# Autodesk Inventor assembly: Tablet-Halterung Nacharbeit
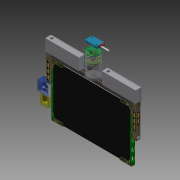
[picture p0: Inventor's stored thumbnail of the model, 180x180]
Saved by Autodesk Inventor 2014 SP1 (Build 180222100, 222)
## iProperties
Created: 2013-08-01
Part Number: Tablet-Halterung Nacharbeit
Document SubType Name: Assembly
Designer: vogel
Author: vogel
## Documents named in this file (59)
- Z:\131087 - Tablet-Halterung\Tablet-Halterung Nacharbeit.iam
- Z:\131087 - Tablet-Halterung\13_1087_001.ipt
- Z:\131087 - Tablet-Halterung\Tablet - Nexus 10.ipt
- Z:\131087 - Tablet-Halterung\13_1087_003.ipt
- Z:\131087 - Tablet-Halterung\13_1087_004.ipt
- C:\Users\vogel.WWF-AD\Documents\Inventor\Content Center Files\R2014\de-DE\ISO 8734(2)\ISO 8734 - 2 x 12 - AISO (2).ipt
- Z:\131087 - Tablet-Halterung\13_1087_005.ipt
- Z:\131087 - Tablet-Halterung\13_1087_002.ipt
- Z:\131087 - Tablet-Halterung\13_1087_007.ipt
- Z:\131087 - Tablet-Halterung\Getriebe.iam
- Z:\131087 - Tablet-Halterung\13_1087_008.ipt
- Z:\131087 - Tablet-Halterung\13_1087_009.ipt
- Z:\131087 - Tablet-Halterung\Sinterbuchse 35 60 325 48106.ipt
- Z:\131087 - Tablet-Halterung\13_1087_016.ipt
- Z:\131087 - Tablet-Halterung\13_1087_017.ipt
- Z:\131087 - Tablet-Halterung\IOIO Board.ipt
- Z:\131087 - Tablet-Halterung\13_1087_018.ipt
- Z:\131087 - Tablet-Halterung\13_1087_019.ipt
- C:\Users\vogel.WWF-AD\Documents\Inventor\Content Center Files\R2014\de-DE\ISO 4026\ISO 4026 - M3 x 5ISO.ipt
- Z:\131087 - Tablet-Halterung\13_1087_020.ipt
- Z:\131087 - Tablet-Halterung\Akku.ipt
- Z:\131087 - Tablet-Halterung\Platine.ipt
- Z:\131087 - Tablet-Halterung\13_0204_040.ipt
- Z:\131087 - Tablet-Halterung\13_1087_023.ipt
- Z:\131087 - Tablet-Halterung\13_1087_024.ipt
- Z:\131087 - Tablet-Halterung\Motor XDRIVE GM12F.ipt
- Z:\131087 - Tablet-Halterung\13_1087_025.ipt
- Z:\131087 - Tablet-Halterung\13_1087_027.ipt
- Z:\131087 - Tablet-Halterung\13_1087_028.ipt
- Z:\131087 - Tablet-Halterung\13_1087_029.ipt
- Z:\131087 - Tablet-Halterung\13_1087_030.ipt
- Z:\131087 - Tablet-Halterung\13_1087_032.ipt
- Z:\131087 - Tablet-Halterung\Sinterbuchse 35 60 325 61014.ipt
- C:\Users\vogel.WWF-AD\Documents\Inventor\Content Center Files\R2014\de-DE\ISO 8734(2)\ISO 8734 - 3 x 8 - AISO (2).ipt
- Z:\131087 - Tablet-Halterung\13_1087_034.ipt
- Z:\131087 - Tablet-Halterung\13_1087_035.ipt
- Z:\131087 - Tablet-Halterung\13_1087_036.ipt
- Z:\131087 - Tablet-Halterung\13_1087_037.ipt
- Z:\131087 - Tablet-Halterung\13_1087_038.ipt
- Z:\131087 - Tablet-Halterung\13_1087_039.ipt
- Z:\131087 - Tablet-Halterung\13_1087_040.ipt
- C:\Users\vogel.WWF-AD\Documents\Inventor\Content Center Files\R2014\de-DE\ISO 2009(2)\ISO 2009 - M2 x 6ISO 4.ipt
- C:\Users\vogel.WWF-AD\Documents\Inventor\Content Center Files\R2014\de-DE\ISO 2009(2)\ISO 2009 - M3 x 6ISO 3,35.ipt
- C:\Users\vogel.WWF-AD\Documents\Inventor\Content Center Files\R2014\de-DE\ISO 10642(1)\ISO 10642 - M3 x  10.ipt
- Z:\131087 - Tablet-Halterung\13_1087_041.ipt
- C:\Users\vogel.WWF-AD\Documents\Inventor\Content Center Files\R2014\de-DE\ISO 2009(2)\ISO 2009 - M2 x 12ISO 10.ipt
- C:\Users\vogel.WWF-AD\Documents\Inventor\Content Center Files\R2014\de-DE\ISO 10642(1)\ISO 10642 - M3 x  16.ipt
- C:\Users\vogel.WWF-AD\Documents\Inventor\Content Center Files\R2014\de-DE\ISO 2009(2)\ISO 2009 - M2 x 3ISO 1.ipt
- C:\Users\vogel.WWF-AD\Documents\Inventor\Content Center Files\R2014\de-DE\ISO 1207(2)\ISO 1207 - M1,6 x 6.ipt
- C:\Users\vogel.WWF-AD\Documents\Inventor\Content Center Files\R2014\de-DE\DIN 6799\DIN 6799 - 2,3 3.ipt
- C:\Users\vogel.WWF-AD\Documents\Inventor\Content Center Files\R2014\de-DE\ISO 4762(2)\ISO 4762 - M4 x 12ISO.ipt
- C:\Users\vogel.WWF-AD\Documents\Inventor\Content Center Files\R2014\de-DE\ISO 4766(1)\ISO 4766 - M2 x 2DIN EN.ipt
- C:\Users\vogel.WWF-AD\Documents\Inventor\Content Center Files\R2014\de-DE\ISO 10642(1)\ISO 10642 - M3 x  8.ipt
- Z:\131087 - Tablet-Halterung\13_1087_042.ipt
- C:\Users\vogel.WWF-AD\Documents\Inventor\Content Center Files\R2014\de-DE\DIN 471(3)\DIN 471 - 4 x 0,4.ipt
- Z:\131087 - Tablet-Halterung\Zahnräder mädler 21401200.ipt
- C:\Users\vogel.WWF-AD\Documents\Inventor\Content Center Files\R2014\de-DE\ISO 4026\ISO 4026 - M3 x 3ISO.ipt
- Z:\131087 - Tablet-Halterung\13_1087_060.ipt
- Z:\131087 - Tablet-Halterung\13_1087_061.ipt
## Components (124 placed, 58 different names)
1. 13_1087_001:1 — Passend:2, Fluchtend:2, Passend:8, Passend:40, Passend:132
2. Tablet - Nexus 10:1 — Passend:2, Passend:5, Passend:9, Passend:10, Fluchtend:7
3. 13_1087_001:2 — Einfügen:2, Passend:11, Passend:130
4. 13_1087_001:3 — Passend:5, Passend:6, Passend:7, Fluchtend:1, Passend:131
5. 13_1087_003:1 — Passend:6, Passend:7, Fluchtend:1, Einfügen:1, Winkel:1, Passend:9, Fluchtend:3, Fluchtend:4, Einfügen:10, Passend:24, Einfügen:12, Passend:39
6. 13_1087_004:1 — Fluchtend:2, Verschiebbar:1, Passend:8, Passend:40
7. 13_1087_005:1 — Passend:10, Fluchtend:3, Fluchtend:4, Einfügen:2, Passend:11, Passend:12, Passend:13, Fluchtend:5, Einfügen:3, Passend:67, Passend:88, Passend:117, Fluchtend:29
8. 13_1087_004:2 — Passend:12, Passend:13, Fluchtend:5, Einfügen:4, Passend:14
9. 13_1087_002:1 — Einfügen:4, Passend:14, Passend:133
10. 13_1087_007:1 — Fluchtend:7, Passend:22, Einfügen:7, Fluchtend:8, Einfügen:14, Passend:59, Passend:94, Passend:95, Passend:102, Passend:103, Passend:104, Passend:105, Passend:115, Passend:116, Achse 1, Einfügen:73, Passend:166
11. 13_1087_016:1 — Passend:24, Einfügen:12, Passend:38, Einfügen:39, Achse 2, Einfügen:72
12. Getriebe:1 [sub-assembly] — Passend:37, Passend:66, Passend:67, Passend:99
13. 13_1087_008:1 — Fluchtend:8, Einfügen:14, Fluchtend:9, Fluchtend:10, Fluchtend:11, Passend:28, Passend:29, Passend:30, Passend:31, Passend:32, Passend:33, Passend:37, Passend:66, Passend:96, Passend:97, Passend:98, Passend:114, Fluchtend:32
14. 13_1087_009:1 — Passend:22, Einfügen:7, Einfügen:8, Passend:34, Passend:35, Passend:36, Achse 2, Passend:41, Passend:42, Passend:43, Passend:44, Passend:45, Passend:46, Fluchtend:21, Passend:107, Passend:108, Passend:109, Einfügen:71, Fluchtend:31
15. Sinterbuchse 35 60 325 48106:1 — Einfügen:8, Einfügen:39
16. 13_1087_017:1 — Einfügen:10, Fluchtend:28
17. IOIO Board:1 — Passend:57, Passend:58, Passend:76
18. 13_1087_018:1 — Fluchtend:9, Passend:28, Passend:29, Passend:122, Passend:123, Einfügen:62, Einfügen:65
19. 13_1087_019:1 — Fluchtend:10, Passend:30, Passend:31, Einfügen:20, Einfügen:23, Passend:120, Passend:121
20. 13_1087_018:2 — Fluchtend:11, Passend:32, Passend:33, Passend:118, Passend:119, Einfügen:60, Einfügen:63
21. 13_1087_018:3 — Passend:34, Passend:35, Passend:36, Einfügen:50, Einfügen:51, Passend:124, Passend:125
22. 13_1087_019:2 — Passend:41, Passend:42, Passend:43, Einfügen:16, Einfügen:17, Passend:126, Passend:127
23. 13_1087_018:4 — Passend:44, Passend:45, Passend:46, Passend:128, Passend:129, Einfügen:58, Einfügen:59
24. Akku:1 — Passend:50, Passend:51, Passend:52
25. 13_1087_017:2 — Passend:88, Fluchtend:28
26. Platine:1 — Passend:54, Passend:77, Passend:78
27. 13_0204_040:1 — Einfügen:43, Einfügen:44, Achse 1
28. 13_1087_023:1 — Fluchtend:15, Fluchtend:16, Passend:49, Passend:50, Passend:51, Passend:52, Fluchtend:20, Fluchtend:21, Fluchtend:22, Fluchtend:32
29. 13_1087_024:1 — Fluchtend:15, Fluchtend:16, Passend:49, Passend:144, Passend:145, Passend:146, Passend:147
30. 13_1087_023:2 — Passend:54, Passend:57, Passend:58, Fluchtend:20, Einfügen:30, Einfügen:31, Passend:59, Fluchtend:22, Passend:76, Passend:77, Passend:78, Passend:91, Passend:92, Passend:93, Fluchtend:31
31. 13_1087_024:2 — Einfügen:30, Einfügen:31, Passend:140, Passend:141, Passend:142, Passend:143
32. Motor XDRIVE GM12F:1 — Einfügen:34, Einfügen:41, Passend:153
33. 13_1087_025:1 — Einfügen:46, Passend:165, Einfügen:76
34. 13_1087_027:1 — Einfügen:34, Passend:72, Passend:154, Passend:159, Passend:160
35. 13_1087_030:1 — Passend:72, Einfügen:41, Einfügen:45, Passend:86, Einfügen:53, Einfügen:54, Einfügen:66, Einfügen:67, Einfügen:74, Passend:167, Passend:168
36. 13_1087_032:1 — Einfügen:43, Einfügen:44, Einfügen:49, Passend:82, Passend:83, Einfügen:52, Fluchtend:26, Passend:84, Einfügen:55, Einfügen:56
37. Sinterbuchse 35 60 325 61014:1 — Einfügen:45, Einfügen:46
38. 13_1087_034:1 — Passend:82, Passend:83
39. 13_1087_035:1 — Einfügen:52, Passend:85, Passend:139
40. 13_1087_036:1 — Fluchtend:26, Passend:84, Passend:85, Passend:155
41. 13_1087_037:1 — Passend:86, Passend:137, Passend:138, Einfügen:66, Einfügen:67
42. 13_1087_038:1 — Passend:91, Passend:92, Passend:93, Passend:100, Passend:101
43. 13_1087_039:1 — Passend:94, Passend:95, Passend:96, Passend:148, Passend:149
44. 13_1087_040:1 — Passend:97, Passend:98, Passend:99, Passend:112, Passend:113
45. 13_1087_041:1 — Passend:107, Passend:108, Passend:109, Passend:110, Passend:111
46. ISO 8734 2 x 12 - A:1 — Einfügen:1, Winkel:1, Verschiebbar:1
47. ISO 8734 2 x 12 - A:2 — Einfügen:3
48. ISO 4026 M3 x 5:1 — Passend:38, Passend:39
49. ISO 8734 3 x 8 - A:1 — Einfügen:49
50. ISO 2009 M2 x 6 x 4:1 — Passend:100
51. ISO 2009 M2 x 6 x 4:2 — Passend:101
52. ISO 2009 M3 x 6 x 3,35:1 — Passend:102
53. ISO 2009 M3 x 6 x 3,35:2 — Passend:103
54. ISO 2009 M3 x 6 x 3,35:3 — Passend:104
55. ISO 2009 M3 x 6 x 3,35:4 — Passend:105
56. ISO 2009 M2 x 12 x 10:1 — Passend:110
57. ISO 2009 M2 x 12 x 10:2 — Passend:111
58. ISO 2009 M2 x 12 x 10:3 — Passend:112
59. ISO 2009 M2 x 12 x 10:4 — Passend:113
60. ISO 10642 M3 x  10:2 — Passend:114
61. ISO 10642 M3 x  16:1 — Passend:115
62. ISO 10642 M3 x  16:2 — Passend:116
63. ISO 4026 M3 x 5:2 — Passend:117, Fluchtend:29
64. ISO 2009 M2 x 3 x 1:1 — Passend:118
65. ISO 2009 M2 x 3 x 1:2 — Passend:119
66. ISO 2009 M2 x 3 x 1:3 — Passend:120
67. ISO 2009 M2 x 3 x 1:4 — Passend:121
68. ISO 2009 M2 x 3 x 1:5 — Passend:122
69. ISO 2009 M2 x 3 x 1:6 — Passend:123
70. ISO 2009 M2 x 3 x 1:7 — Passend:124
71. ISO 2009 M2 x 3 x 1:8 — Passend:125
72. ISO 2009 M2 x 3 x 1:9 — Passend:126
73. ISO 2009 M2 x 3 x 1:10 — Passend:127
74. ISO 2009 M2 x 3 x 1:11 — Passend:128
75. ISO 2009 M2 x 3 x 1:12 — Passend:129
76. ISO 2009 M2 x 6 x 4:3 — Passend:130
77. ISO 2009 M2 x 6 x 4:4 — Passend:131
78. ISO 2009 M2 x 6 x 4:5 — Passend:132
79. ISO 2009 M2 x 6 x 4:6 — Passend:133
80. ISO 10642 M3 x  10:3 — Passend:137
81. ISO 10642 M3 x  10:4 — Passend:138
82. ISO 1207 M1,6 x 6:1 — Einfügen:53
83. ISO 1207 M1,6 x 6:2 — Einfügen:54
84. DIN 6799 2,3:1 — Passend:139
85. ISO 4762 M4 x 12:1 — Einfügen:55
86. ISO 4762 M4 x 12:2 — Einfügen:56
87. ISO 2009 M2 x 6 x 4:7 — Passend:140
88. ISO 2009 M2 x 6 x 4:8 — Passend:141
89. ISO 2009 M2 x 6 x 4:9 — Passend:142
90. ISO 2009 M2 x 6 x 4:10 — Passend:143
91. ISO 2009 M2 x 6 x 4:11 — Passend:144
92. ISO 2009 M2 x 6 x 4:12 — Passend:145
93. ISO 2009 M2 x 6 x 4:13 — Passend:146
94. ISO 2009 M2 x 6 x 4:14 — Passend:147
95. ISO 2009 M2 x 12 x 10:5 — Passend:148
96. ISO 2009 M2 x 12 x 10:6 — Passend:149
97. DIN EN 24766 M2 x 2:1 — Passend:153, Passend:154
98. ISO 10642 M3 x  8:1 — Passend:155
99. 13_1087_042:1 — Einfügen:71
100. DIN 471 <= 9mm 4 x 0,4:1 — Einfügen:72
101. Zahnräder mädler 21401200:1 — Passend:159, Passend:160, Fluchtend:30, Passend:161, Passend:162
102. Zahnräder mädler 21401200:2 — Fluchtend:30, Passend:163, Passend:164, Passend:165
103. ISO 4026 M3 x 3:1 — Passend:161, Passend:162
104. ISO 4026 M3 x 3:2 — Passend:163, Passend:164
105. 13_1087_060:1 — Einfügen:73, Passend:166, Einfügen:74, Passend:167, Einfügen:75
106. 13_1087_028:1 — Einfügen:76, Einfügen:77
107. 13_1087_029:1 — Einfügen:75, Passend:168
108. 13_1087_061:1 — Einfügen:77
109. 13_1087_020:3 — Einfügen:20, Einfügen:23
110. 13_1087_020:9
111. 13_1087_020:5 — Einfügen:16, Einfügen:17
112. 13_1087_020:14
113. 13_1087_020:22 — Einfügen:62, Einfügen:65
114. 13_1087_020:20 — Einfügen:60, Einfügen:63
115. 13_1087_020:19 — Einfügen:58, Einfügen:59
116. 13_1087_020:17 — Einfügen:50, Einfügen:51
117. 13_1087_020:25
118. 13_1087_020:26
119. 13_1087_020:27
120. 13_1087_020:28
121. 13_1087_020:29
122. 13_1087_020:30
123. 13_1087_020:31
124. 13_1087_020:32
## Component patterns: (2 elements, first: 13_1087_020:3), (2 elements, first: 13_1087_020:5), (3 elements, first: 13_1087_020:22 + 13_1087_020:20 + 13_1087_020:19 + 13_1087_020:17)
## Relationships (190: Mate 120, Insert 45, Flush 21, Angle 3, TranslationJoint 1)
- Passend:2 [Mate]: 13_1087_001:1 ↔ Tablet - Nexus 10:1
- Passend:5 [Mate]: Tablet - Nexus 10:1 ↔ 13_1087_001:3
- Passend:6 [Mate]: 13_1087_001:3 ↔ 13_1087_003:1
- Passend:7 [Mate]: 13_1087_001:3 ↔ 13_1087_003:1
- Fluchtend:1 [Flush]: 13_1087_001:3 ↔ 13_1087_003:1
- Fluchtend:2 [Flush]: 13_1087_001:1 ↔ 13_1087_004:1
- Einfügen:1 [Insert]: 13_1087_003:1 ↔ ISO 8734 2 x 12 - A:1
- Winkel:1 [Angle] (90 deg): 13_1087_003:1 ↔ ISO 8734 2 x 12 - A:1
- Verschiebbar:1 [TranslationJoint]: 13_1087_004:1 ↔ ISO 8734 2 x 12 - A:1
- Passend:8 [Mate]: 13_1087_001:1 ↔ 13_1087_004:1
- Passend:9 [Mate] (0.1 mm): Tablet - Nexus 10:1 ↔ 13_1087_003:1
- Passend:10 [Mate] (0.1 mm): Tablet - Nexus 10:1 ↔ 13_1087_005:1
- Fluchtend:3 [Flush]: 13_1087_003:1 ↔ 13_1087_005:1
- Fluchtend:4 [Flush]: 13_1087_003:1 ↔ 13_1087_005:1
- Einfügen:2 [Insert]: 13_1087_001:2 ↔ 13_1087_005:1
- Passend:11 [Mate]: 13_1087_001:2 ↔ 13_1087_005:1
- Passend:12 [Mate]: 13_1087_005:1 ↔ 13_1087_004:2
- Passend:13 [Mate]: 13_1087_005:1 ↔ 13_1087_004:2
- Fluchtend:5 [Flush]: 13_1087_005:1 ↔ 13_1087_004:2
- Einfügen:3 [Insert]: 13_1087_005:1 ↔ ISO 8734 2 x 12 - A:2
- Einfügen:4 [Insert]: 13_1087_004:2 ↔ 13_1087_002:1
- Passend:14 [Mate]: 13_1087_004:2 ↔ 13_1087_002:1
- Fluchtend:7 [Flush]: Tablet - Nexus 10:1 ↔ 13_1087_007:1
- Passend:22 [Mate]: 13_1087_007:1 ↔ 13_1087_009:1
- Einfügen:7 [Insert]: 13_1087_007:1 ↔ 13_1087_009:1
- Einfügen:8 [Insert]: 13_1087_009:1 ↔ Sinterbuchse 35 60 325 48106:1
- Einfügen:10 [Insert]: 13_1087_003:1 ↔ 13_1087_017:1
- Passend:24 [Mate]: 13_1087_003:1 ↔ 13_1087_016:1
- Einfügen:12 [Insert] (1.5 mm): 13_1087_003:1 ↔ 13_1087_016:1
- Fluchtend:8 [Flush]: 13_1087_007:1 ↔ 13_1087_008:1
- Einfügen:14 [Insert]: 13_1087_007:1 ↔ 13_1087_008:1
- Fluchtend:9 [Flush] (-3.5 mm): 13_1087_008:1 ↔ 13_1087_018:1
- Fluchtend:10 [Flush] (3.5 mm): 13_1087_008:1 ↔ 13_1087_019:1
- Fluchtend:11 [Flush] (-3.5 mm): 13_1087_008:1 ↔ 13_1087_018:2
- Passend:28 [Mate]: 13_1087_008:1 ↔ 13_1087_018:1
- Passend:29 [Mate]: 13_1087_008:1 ↔ 13_1087_018:1
- Passend:30 [Mate]: 13_1087_008:1 ↔ 13_1087_019:1
- Passend:31 [Mate]: 13_1087_008:1 ↔ 13_1087_019:1
- Passend:32 [Mate]: 13_1087_008:1 ↔ 13_1087_018:2
- Passend:33 [Mate]: 13_1087_008:1 ↔ 13_1087_018:2
- Passend:34 [Mate]: 13_1087_009:1 ↔ 13_1087_018:3
- Passend:35 [Mate]: 13_1087_009:1 ↔ 13_1087_018:3
- Passend:36 [Mate]: 13_1087_009:1 ↔ 13_1087_018:3
- Passend:37 [Mate]: Getriebe:1 ↔ 13_1087_008:1
- Passend:38 [Mate]: 13_1087_016:1 ↔ ISO 4026 M3 x 5:1
- Passend:39 [Mate]: 13_1087_003:1 ↔ ISO 4026 M3 x 5:1
- Passend:40 [Mate]: 13_1087_001:1 ↔ 13_1087_004:1
- Passend:41 [Mate]: 13_1087_009:1 ↔ 13_1087_019:2
- Passend:42 [Mate]: 13_1087_009:1 ↔ 13_1087_019:2
- Passend:43 [Mate]: 13_1087_009:1 ↔ 13_1087_019:2
- Passend:44 [Mate]: 13_1087_009:1 ↔ 13_1087_018:4
- Passend:45 [Mate]: 13_1087_009:1 ↔ 13_1087_018:4
- Passend:46 [Mate]: 13_1087_009:1 ↔ 13_1087_018:4
- Einfügen:16 [Insert]: 13_1087_019:2 ↔ 13_1087_020:5
- Einfügen:17 [Insert]: 13_1087_019:2 ↔ 13_1087_020:5
- Einfügen:20 [Insert]: 13_1087_019:1 ↔ 13_1087_020:3
- Einfügen:23 [Insert]: 13_1087_019:1 ↔ 13_1087_020:3
- Fluchtend:15 [Flush]: 13_1087_023:1 ↔ 13_1087_024:1
- Fluchtend:16 [Flush]: 13_1087_023:1 ↔ 13_1087_024:1
- Passend:49 [Mate]: 13_1087_023:1 ↔ 13_1087_024:1
- Passend:50 [Mate]: Akku:1 ↔ 13_1087_023:1
- Passend:51 [Mate]: Akku:1 ↔ 13_1087_023:1
- Passend:52 [Mate]: Akku:1 ↔ 13_1087_023:1
- Passend:54 [Mate] (4 mm): Platine:1 ↔ 13_1087_023:2
- Passend:57 [Mate] (4 mm): IOIO Board:1 ↔ 13_1087_023:2
- Passend:58 [Mate] (5 mm): IOIO Board:1 ↔ 13_1087_023:2
- Fluchtend:20 [Flush]: 13_1087_023:1 ↔ 13_1087_023:2
- Einfügen:30 [Insert]: 13_1087_023:2 ↔ 13_1087_024:2
- Einfügen:31 [Insert]: 13_1087_023:2 ↔ 13_1087_024:2
- Passend:59 [Mate]: 13_1087_007:1 ↔ 13_1087_023:2
- Fluchtend:21 [Flush] (-3 mm): 13_1087_009:1 ↔ 13_1087_023:1
- Fluchtend:22 [Flush]: 13_1087_023:1 ↔ 13_1087_023:2
- Passend:66 [Mate]: Getriebe:1 ↔ 13_1087_008:1
- Passend:67 [Mate]: 13_1087_005:1 ↔ Getriebe:1
- Einfügen:34 [Insert] (-3.5 mm): Motor XDRIVE GM12F:1 ↔ 13_1087_027:1
- Passend:72 [Mate]: 13_1087_027:1 ↔ 13_1087_030:1
- Einfügen:39 [Insert]: 13_1087_016:1 ↔ Sinterbuchse 35 60 325 48106:1
- Achse 2 [Angle] (180 deg): 13_1087_016:1 ↔ 13_1087_009:1
- Einfügen:41 [Insert]: Motor XDRIVE GM12F:1 ↔ 13_1087_030:1
- Einfügen:43 [Insert]: 13_0204_040:1 ↔ 13_1087_032:1
- Einfügen:44 [Insert]: 13_0204_040:1 ↔ 13_1087_032:1
- Passend:76 [Mate] (2.5 mm): IOIO Board:1 ↔ 13_1087_023:2
- Passend:77 [Mate]: Platine:1 ↔ 13_1087_023:2
- Passend:78 [Mate] (5 mm): Platine:1 ↔ 13_1087_023:2
- Einfügen:45 [Insert]: 13_1087_030:1 ↔ Sinterbuchse 35 60 325 61014:1
- Einfügen:46 [Insert]: 13_1087_025:1 ↔ Sinterbuchse 35 60 325 61014:1
- Einfügen:49 [Insert]: 13_1087_032:1 ↔ ISO 8734 3 x 8 - A:1
- Einfügen:50 [Insert]: 13_1087_018:3 ↔ 13_1087_020:17
- Einfügen:51 [Insert]: 13_1087_018:3 ↔ 13_1087_020:17
- Passend:82 [Mate]: 13_1087_032:1 ↔ 13_1087_034:1
- Passend:83 [Mate]: 13_1087_032:1 ↔ 13_1087_034:1
- Einfügen:52 [Insert]: 13_1087_032:1 ↔ 13_1087_035:1
- Fluchtend:26 [Flush]: 13_1087_032:1 ↔ 13_1087_036:1
- Passend:84 [Mate]: 13_1087_032:1 ↔ 13_1087_036:1
- Passend:85 [Mate]: 13_1087_035:1 ↔ 13_1087_036:1
- Passend:86 [Mate]: 13_1087_030:1 ↔ 13_1087_037:1
- Passend:88 [Mate]: 13_1087_005:1 ↔ 13_1087_017:2
- Fluchtend:28 [Flush]: 13_1087_017:1 ↔ 13_1087_017:2
- Passend:91 [Mate]: 13_1087_023:2 ↔ 13_1087_038:1
- Passend:92 [Mate] (0.5 mm): 13_1087_023:2 ↔ 13_1087_038:1
- Passend:93 [Mate] (0.5 mm): 13_1087_023:2 ↔ 13_1087_038:1
- Passend:94 [Mate]: 13_1087_007:1 ↔ 13_1087_039:1
- Passend:95 [Mate]: 13_1087_007:1 ↔ 13_1087_039:1
- Passend:96 [Mate] (1 mm): 13_1087_008:1 ↔ 13_1087_039:1
- Passend:97 [Mate]: 13_1087_008:1 ↔ 13_1087_040:1
- Passend:98 [Mate]: 13_1087_008:1 ↔ 13_1087_040:1
- Passend:99 [Mate]: Getriebe:1 ↔ 13_1087_040:1
- Passend:100 [Mate]: 13_1087_038:1 ↔ ISO 2009 M2 x 6 x 4:1
- Passend:101 [Mate]: 13_1087_038:1 ↔ ISO 2009 M2 x 6 x 4:2
- Passend:102 [Mate]: 13_1087_007:1 ↔ ISO 2009 M3 x 6 x 3,35:1
- Passend:103 [Mate]: 13_1087_007:1 ↔ ISO 2009 M3 x 6 x 3,35:2
- Passend:104 [Mate]: 13_1087_007:1 ↔ ISO 2009 M3 x 6 x 3,35:3
- Passend:105 [Mate]: 13_1087_007:1 ↔ ISO 2009 M3 x 6 x 3,35:4
- Passend:107 [Mate]: 13_1087_009:1 ↔ 13_1087_041:1
- Passend:108 [Mate]: 13_1087_009:1 ↔ 13_1087_041:1
- Passend:109 [Mate]: 13_1087_009:1 ↔ 13_1087_041:1
- Passend:110 [Mate]: 13_1087_041:1 ↔ ISO 2009 M2 x 12 x 10:1
- Passend:111 [Mate]: 13_1087_041:1 ↔ ISO 2009 M2 x 12 x 10:2
- Passend:112 [Mate]: 13_1087_040:1 ↔ ISO 2009 M2 x 12 x 10:3
- Passend:113 [Mate]: 13_1087_040:1 ↔ ISO 2009 M2 x 12 x 10:4
- Passend:114 [Mate]: 13_1087_008:1 ↔ ISO 10642 M3 x  10:2
- Passend:115 [Mate]: 13_1087_007:1 ↔ ISO 10642 M3 x  16:1
- Passend:116 [Mate]: 13_1087_007:1 ↔ ISO 10642 M3 x  16:2
- Passend:117 [Mate]: 13_1087_005:1 ↔ ISO 4026 M3 x 5:2
- Fluchtend:29 [Flush]: 13_1087_005:1 ↔ ISO 4026 M3 x 5:2
- Passend:118 [Mate]: 13_1087_018:2 ↔ ISO 2009 M2 x 3 x 1:1
- Passend:119 [Mate]: 13_1087_018:2 ↔ ISO 2009 M2 x 3 x 1:2
- Passend:120 [Mate]: 13_1087_019:1 ↔ ISO 2009 M2 x 3 x 1:3
- Passend:121 [Mate]: 13_1087_019:1 ↔ ISO 2009 M2 x 3 x 1:4
- Passend:122 [Mate]: 13_1087_018:1 ↔ ISO 2009 M2 x 3 x 1:5
- Passend:123 [Mate]: 13_1087_018:1 ↔ ISO 2009 M2 x 3 x 1:6
- Passend:124 [Mate]: 13_1087_018:3 ↔ ISO 2009 M2 x 3 x 1:7
- Passend:125 [Mate]: 13_1087_018:3 ↔ ISO 2009 M2 x 3 x 1:8
- Passend:126 [Mate]: 13_1087_019:2 ↔ ISO 2009 M2 x 3 x 1:9
- Passend:127 [Mate]: 13_1087_019:2 ↔ ISO 2009 M2 x 3 x 1:10
- Passend:128 [Mate]: 13_1087_018:4 ↔ ISO 2009 M2 x 3 x 1:11
- Passend:129 [Mate]: 13_1087_018:4 ↔ ISO 2009 M2 x 3 x 1:12
- Passend:130 [Mate]: 13_1087_001:2 ↔ ISO 2009 M2 x 6 x 4:3
- Passend:131 [Mate]: 13_1087_001:3 ↔ ISO 2009 M2 x 6 x 4:4
- Passend:132 [Mate]: 13_1087_001:1 ↔ ISO 2009 M2 x 6 x 4:5
- Passend:133 [Mate]: 13_1087_002:1 ↔ ISO 2009 M2 x 6 x 4:6
- Passend:137 [Mate]: 13_1087_037:1 ↔ ISO 10642 M3 x  10:3
- Passend:138 [Mate]: 13_1087_037:1 ↔ ISO 10642 M3 x  10:4
- Einfügen:53 [Insert]: 13_1087_030:1 ↔ ISO 1207 M1,6 x 6:1
- Einfügen:54 [Insert]: 13_1087_030:1 ↔ ISO 1207 M1,6 x 6:2
- Passend:139 [Mate]: 13_1087_035:1 ↔ DIN 6799 2,3:1
- Einfügen:55 [Insert]: 13_1087_032:1 ↔ ISO 4762 M4 x 12:1
- Einfügen:56 [Insert]: 13_1087_032:1 ↔ ISO 4762 M4 x 12:2
- Passend:140 [Mate]: 13_1087_024:2 ↔ ISO 2009 M2 x 6 x 4:7
- Passend:141 [Mate]: 13_1087_024:2 ↔ ISO 2009 M2 x 6 x 4:8
- Passend:142 [Mate]: 13_1087_024:2 ↔ ISO 2009 M2 x 6 x 4:9
- Passend:143 [Mate]: 13_1087_024:2 ↔ ISO 2009 M2 x 6 x 4:10
- Passend:144 [Mate]: 13_1087_024:1 ↔ ISO 2009 M2 x 6 x 4:11
- Passend:145 [Mate]: 13_1087_024:1 ↔ ISO 2009 M2 x 6 x 4:12
- Passend:146 [Mate]: 13_1087_024:1 ↔ ISO 2009 M2 x 6 x 4:13
- Passend:147 [Mate]: 13_1087_024:1 ↔ ISO 2009 M2 x 6 x 4:14
- Passend:148 [Mate]: 13_1087_039:1 ↔ ISO 2009 M2 x 12 x 10:5
- Passend:149 [Mate]: 13_1087_039:1 ↔ ISO 2009 M2 x 12 x 10:6
- Einfügen:58 [Insert]: 13_1087_018:4 ↔ 13_1087_020:19
- Einfügen:59 [Insert]: 13_1087_018:4 ↔ 13_1087_020:19
- Einfügen:60 [Insert]: 13_1087_018:2 ↔ 13_1087_020:20
- Einfügen:62 [Insert]: 13_1087_018:1 ↔ 13_1087_020:22
- Einfügen:63 [Insert]: 13_1087_018:2 ↔ 13_1087_020:20
- Einfügen:65 [Insert]: 13_1087_018:1 ↔ 13_1087_020:22
- Passend:153 [Mate]: Motor XDRIVE GM12F:1 ↔ DIN EN 24766 M2 x 2:1
- Passend:154 [Mate]: 13_1087_027:1 ↔ DIN EN 24766 M2 x 2:1
- Passend:155 [Mate]: 13_1087_036:1 ↔ ISO 10642 M3 x  8:1
- Einfügen:66 [Insert]: 13_1087_030:1 ↔ 13_1087_037:1
- Einfügen:67 [Insert]: 13_1087_030:1 ↔ 13_1087_037:1
- Achse 1 [Angle] (0 deg): 13_1087_007:1 ↔ 13_0204_040:1
- Einfügen:71 [Insert]: 13_1087_009:1 ↔ 13_1087_042:1
- Einfügen:72 [Insert]: 13_1087_016:1 ↔ DIN 471 <= 9mm 4 x 0,4:1
- Passend:159 [Mate]: 13_1087_027:1 ↔ Zahnräder mädler 21401200:1
- Passend:160 [Mate] (2 mm): 13_1087_027:1 ↔ Zahnräder mädler 21401200:1
- Fluchtend:30 [Flush]: Zahnräder mädler 21401200:1 ↔ Zahnräder mädler 21401200:2
- Passend:161 [Mate]: Zahnräder mädler 21401200:1 ↔ ISO 4026 M3 x 3:1
- Passend:162 [Mate] (2.5 mm): Zahnräder mädler 21401200:1 ↔ ISO 4026 M3 x 3:1
- Passend:163 [Mate]: Zahnräder mädler 21401200:2 ↔ ISO 4026 M3 x 3:2
- Passend:164 [Mate] (2.5 mm): Zahnräder mädler 21401200:2 ↔ ISO 4026 M3 x 3:2
- Passend:165 [Mate]: 13_1087_025:1 ↔ Zahnräder mädler 21401200:2
- Fluchtend:31 [Flush]: 13_1087_009:1 ↔ 13_1087_023:2
- Fluchtend:32 [Flush]: 13_1087_008:1 ↔ 13_1087_023:1
- Einfügen:73 [Insert]: 13_1087_007:1 ↔ 13_1087_060:1
- Passend:166 [Mate]: 13_1087_007:1 ↔ 13_1087_060:1
- Einfügen:74 [Insert] (-4 mm): 13_1087_030:1 ↔ 13_1087_060:1
- Passend:167 [Mate]: 13_1087_030:1 ↔ 13_1087_060:1
- Einfügen:75 [Insert]: 13_1087_060:1 ↔ 13_1087_029:1
- Passend:168 [Mate]: 13_1087_030:1 ↔ 13_1087_029:1
- Einfügen:76 [Insert] (4 mm): 13_1087_025:1 ↔ 13_1087_028:1
- Einfügen:77 [Insert]: 13_1087_028:1 ↔ 13_1087_061:1
